# Autodesk Inventor assembly: Longhouse
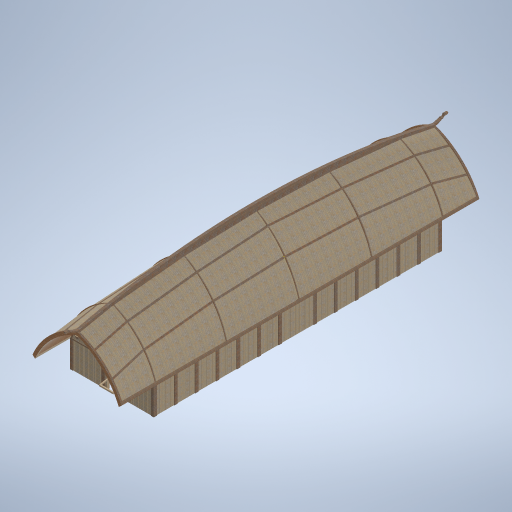
[picture p0: Inventor's stored thumbnail of the model, 512x512]
Saved by Autodesk Inventor 2024.3 (Build 283343000, 343)
## iProperties
Created: 2024-05-22
Part Number: Longhouse
Document SubType Name: Assembly
Designer: LOSTER_1
Author: LOSTER_1
## Documents named in this file (4)
- C:\Users\Huang\OneDrive\桌面\school\senior\Inventor_Project\Longhouse.iam
- C:\Users\Huang\OneDrive\桌面\school\senior\Inventor_Project\ROOF\Roof.iam
- C:\Users\Huang\OneDrive\桌面\school\senior\Inventor_Project\WALL\WallBody.iam
- C:\Users\Huang\OneDrive\桌面\school\senior\Inventor_Project\ROOF\side_eave_parts\eave_frame_01.ipt
## Components (3 placed, 3 different names)
1. Roof:1 [sub-assembly] — Mate:1
2. WallBody:1 [sub-assembly] — Mate:1, Mate:2, Mate:3
3. eave_frame_01:1 — Mate:2, Mate:3
## Relationships (3: Mate 3)
- Mate:1: Roof:1 ↔ WallBody:1
- Mate:2: WallBody:1 ↔ eave_frame_01:1
- Mate:3: WallBody:1 ↔ eave_frame_01:1
